# Autodesk Inventor assembly: ASY GnG station
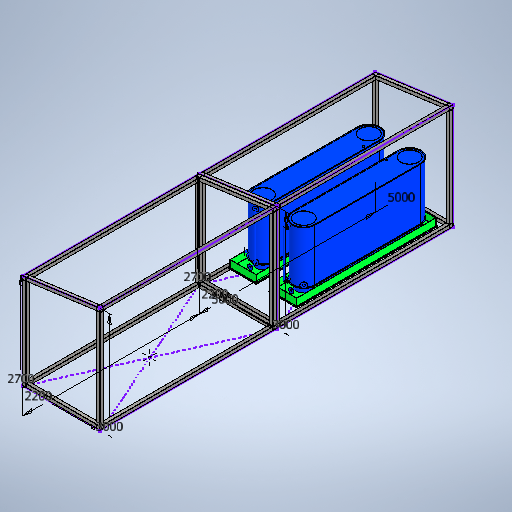
[picture p0: Inventor's stored thumbnail of the model, 512x512]
Saved by Autodesk Inventor 2025 (Build 290162010, 162A)
## iProperties
Created: 2025-09-20
Part Number: ASY GnG station
Document SubType Name: Assembly
Designer: admin
Mass: 766899 g
Surface Area: 646346 cm^2
Volume: 96834.3 cm^3
Density: 7.91971 g/cm^3
Author: admin
## Documents named in this file (5)
- C:\Users\admin\Yandex.Disk\home pc\Inventor\GnG_Gantul_hill\ASY GnG station.iam
- C:\Users\admin\Yandex.Disk\home pc\Inventor\GnG_Gantul_hill\AST GnG frame.iam
- C:\Users\admin\Yandex.Disk\home pc\Inventor\GnG_Gantul_hill\GNG НаOCl pan.ipt
- C:\Users\admin\Yandex.Disk\home pc\Inventor\GnG_Gantul_hill\GNG НаOCl tank 2.ipt
- C:\Users\admin\Yandex.Disk\home pc\Inventor\GnG_Gantul_hill\GNG НаOCl tank 2_MIR.ipt
## Components (6 placed, 4 different names)
1. AST GnG frame:1 [sub-assembly] — Mate:1, Mate:2, Mate:7, Mate:8, Rigid:1
2. GNG НаOCl pan:1 — Mate:2, Mate:6, Flush:2, Mate:8, Tangent:1, Mate:9
3. GNG НаOCl pan:2 — Mate:1, Flush:2, Mate:7
4. GNG НаOCl tank 2:1 — Mate:6, Tangent:1, Mate:9
5. AST GnG frame:2 [sub-assembly] — Rigid:1
6. GNG НаOCl tank 2_MIR:1
## Relationships (9: Mate 6, Flush 1, Tangent 1, WeldJoint 1)
- Mate:1: AST GnG frame:1 ↔ GNG НаOCl pan:2
- Mate:2: AST GnG frame:1 ↔ GNG НаOCl pan:1
- Mate:6 (40 mm): GNG НаOCl pan:1 ↔ GNG НаOCl tank 2:1
- Flush:2: GNG НаOCl pan:1 ↔ GNG НаOCl pan:2
- Mate:7 (25 mm): AST GnG frame:1 ↔ GNG НаOCl pan:2
- Mate:8 (25 mm): AST GnG frame:1 ↔ GNG НаOCl pan:1
- Tangent:1 (50 mm): GNG НаOCl pan:1 ↔ GNG НаOCl tank 2:1
- Mate:9: GNG НаOCl pan:1 ↔ GNG НаOCl tank 2:1
- Rigid:1 [WeldJoint]: AST GnG frame:1 ↔ AST GnG frame:2
